# Autodesk Inventor assembly: ShooterAssembly_NERDS
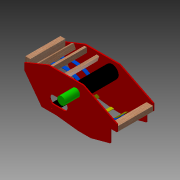
[picture p0: Inventor's stored thumbnail of the model, 180x180]
Saved by Autodesk Inventor 2014 (Build 180170000, 170)
## iProperties
Created: 2016-01-30
Part Number: ShooterAssembly_NERDS
Document SubType Name: Assembly
Designer: bermudezr
Author: bermudezr
## Documents named in this file (13)
- Z:\Nerds_1726\Models\2015-2016\Assemblies\Robot\Shooter.iam
- Z:\Nerds_1726\Models\2015-2016\Parts\Robot\Shooter\ShooterMountLeft.ipt
- Z:\Nerds_1726\Models\2015-2016\Parts\Robot\Shooter\ShooterMountRight.ipt
- Z:\Nerds_1726\Models\2015-2016\Parts\Robot\Shooter\ShootingMotor.ipt
- Z:\Nerds_1726\Models\2015-2016\Parts\Robot\Shooter\LoaderMotor.ipt
- Z:\Nerds_1726\Models\2015-2016\Parts\Robot\Shooter\LoadingRail.ipt
- Z:\Nerds_1726\Models\2015-2016\Parts\Robot\Shooter\ShootingRail.ipt
- Z:\Nerds_1726\Models\2015-2016\Parts\Robot\Shooter\SmallMotor.ipt
- Z:\Nerds_1726\Models\2015-2016\Parts\Robot\Chassis\DriveMotor.ipt
- Z:\Nerds_1726\Models\2015-2016\Parts\Robot\Shooter\RailMount1x2.ipt
- Z:\Nerds_1726\Models\2015-2016\Parts\Robot\Shooter\RailMountMetal.ipt
- Z:\Nerds_1726\Models\2015-2016\Parts\Robot\Shooter\ShieldMount2x4.ipt
- Z:\Nerds_1726\Models\2015-2016\Parts\Robot\Shooter\ShooterFrontMount.ipt
## Components (20 placed, 12 different names)
1. ShooterMountLeft:1 — Flush:2, Mate:1, Mate:2, Mate:5, Mate:25, Mate:26, Flush:8, Mate:27, Mate:28, Flush:9, Mate:29
2. ShooterMountRight:1 — Flush:2, Mate:1, Mate:3, Mate:12, Mate:14, Insert:2, Mate:17, Mate:18, Mate:20, Mate:21, Mate:22, Mate:23, Mate:24, Flush:6, Flush:7
3. ShootingMotor:1 — Mate:2, Mate:5, Mate:9, Mate:10
4. LoaderMotor:1 — Mate:3, Mate:6, Mate:7, Mate:13, Flush:9, Mate:30
5. LoadingRail:1 — Mate:6, Mate:8, Flush:3, Flush:5, Tangent:1, Tangent:2, Tangent:9
6. LoadingRail:2 — Mate:7, Mate:8, Flush:5, Mate:12, Tangent:4
7. ShootingRail:1 — Mate:9, Mate:11, Flush:4, Mate:14, Tangent:7
8. ShootingRail:2 — Mate:10, Mate:11, Flush:3, Flush:4, Mate:13, Tangent:5, Tangent:6, Tangent:8
9. SmallMotor:1 — Mate:29, Mate:30
10. DriveMotor:1 — Insert:2
11. RailMount1x2:1 — Mate:17, Tangent:1
12. RailMount1x2:2 — Mate:18, Tangent:2
13. RailMount1x2:4 — Mate:20, Tangent:4
14. RailMountMetal:1 — Mate:21, Tangent:7
15. RailMountMetal:2 — Mate:22, Tangent:6
16. RailMountMetal:3 — Mate:23, Tangent:5
17. RailMountMetal:4 — Mate:24, Tangent:8
18. ShieldMount2x4:2 — Flush:6, Mate:25, Flush:7
19. ShooterFrontMount:1 — Mate:26, Flush:8, Mate:27
20. RailMountMetal:5 — Mate:28, Tangent:9
## Relationships (43: Mate 26, Flush 8, Tangent 8, Insert 1)
- Flush:2: ShooterMountLeft:1 ↔ ShooterMountRight:1
- Mate:1 (275.8186 mm): ShooterMountLeft:1 ↔ ShooterMountRight:1
- Mate:2: ShooterMountLeft:1 ↔ ShootingMotor:1
- Mate:3: ShooterMountRight:1 ↔ LoaderMotor:1
- Mate:5: ShooterMountLeft:1 ↔ ShootingMotor:1
- Mate:6: LoaderMotor:1 ↔ LoadingRail:1
- Mate:7: LoaderMotor:1 ↔ LoadingRail:2
- Mate:8 (50.8 mm): LoadingRail:1 ↔ LoadingRail:2
- Mate:9: ShootingMotor:1 ↔ ShootingRail:1
- Mate:10: ShootingMotor:1 ↔ ShootingRail:2
- Mate:11 (50.8 mm): ShootingRail:1 ↔ ShootingRail:2
- Flush:3: LoadingRail:1 ↔ ShootingRail:2
- Flush:4: ShootingRail:1 ↔ ShootingRail:2
- Flush:5: LoadingRail:1 ↔ LoadingRail:2
- Mate:12: ShooterMountRight:1 ↔ LoadingRail:2
- Mate:13 (38.1 mm): LoaderMotor:1 ↔ ShootingRail:2
- Mate:14 (76.2 mm): ShooterMountRight:1 ↔ ShootingRail:1
- Insert:2: ShooterMountRight:1 ↔ DriveMotor:1
- Mate:17: ShooterMountRight:1 ↔ RailMount1x2:1
- Tangent:1: LoadingRail:1 ↔ RailMount1x2:1
- Mate:18: ShooterMountRight:1 ↔ RailMount1x2:2
- Mate:20: ShooterMountRight:1 ↔ RailMount1x2:4
- Tangent:2: LoadingRail:1 ↔ RailMount1x2:2
- Tangent:4: LoadingRail:2 ↔ RailMount1x2:4
- Mate:21: ShooterMountRight:1 ↔ RailMountMetal:1
- Mate:22: ShooterMountRight:1 ↔ RailMountMetal:2
- Mate:23: ShooterMountRight:1 ↔ RailMountMetal:3
- Tangent:5: ShootingRail:2 ↔ RailMountMetal:3
- Tangent:6: ShootingRail:2 ↔ RailMountMetal:2
- Tangent:7: ShootingRail:1 ↔ RailMountMetal:1
- Mate:24: ShooterMountRight:1 ↔ RailMountMetal:4
- Tangent:8: ShootingRail:2 ↔ RailMountMetal:4
- Flush:6: ShooterMountRight:1 ↔ ShieldMount2x4:2
- Mate:25: ShooterMountLeft:1 ↔ ShieldMount2x4:2
- Flush:7: ShooterMountRight:1 ↔ ShieldMount2x4:2
- Mate:26: ShooterMountLeft:1 ↔ ShooterFrontMount:1
- Flush:8: ShooterMountLeft:1 ↔ ShooterFrontMount:1
- Mate:27: ShooterMountLeft:1 ↔ ShooterFrontMount:1
- Mate:28: ShooterMountLeft:1 ↔ RailMountMetal:5
- Tangent:9: LoadingRail:1 ↔ RailMountMetal:5
- Flush:9: ShooterMountLeft:1 ↔ LoaderMotor:1
- Mate:29: ShooterMountLeft:1 ↔ SmallMotor:1
- Mate:30: LoaderMotor:1 ↔ SmallMotor:1
